# Autodesk Inventor assembly: M - Climber
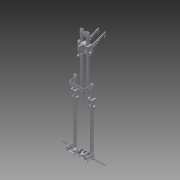
[picture p0: Inventor's stored thumbnail of the model, 180x180]
Saved by Autodesk Inventor 2013 (Build 170138000, 138)
## iProperties
Created: 2013-02-17
Part Number: M - Climber
Document SubType Name: Assembly
Designer: Moses
Mass: 5405.91 g
Surface Area: 9929.51 cm^2
Volume: 1509.49 cm^3
Density: 3.58127 g/cm^3
Author: Moses
## Documents named in this file (6)
- C:\Users\Moses\Documents\GitHub\frc2013CAD\M-Climber\M - Climber.iam
- C:\Users\Moses\Documents\GitHub\frc2013CAD\M-Climber\M - Climber Lower Rails.iam
- C:\Users\Moses\Documents\GitHub\frc2013CAD\M-Climber\M - Climber Upper Rails.iam
- C:\Users\Moses\Documents\GitHub\frc2013CAD\M-Climber\M - Carriage.iam
- C:\Users\Moses\Documents\GitHub\frc2013CAD\M-Climber\rough pulley.ipt
- C:\Users\Moses\Documents\GitHub\frc2013CAD\M-Climber\M - 18 inch shaft.ipt
## Components (8 placed, 5 different names)
1. M - Climber Lower Rails:1 [sub-assembly] — Mate:1, Flush:1, Mate:2, Tangent:1, Tangent:2, Mate:3, Tangent:3, Tangent:4, Mate:4, Mate:5, Flush:4, Mate:9
2. M - Climber Upper Rails:1 [sub-assembly] — Mate:1, Flush:1, Flush:3, Flush:6, Flush:7
3. M - Carriage:1 [sub-assembly] — Mate:2, Tangent:1, Tangent:2, Flush:2, Flush:3, Mate:9
4. M - Carriage:2 [sub-assembly] — Flush:2, Mate:3, Tangent:3, Tangent:4
5. M - 18 inch shaft:1 — Mate:4, Mate:5, Flush:4, Mate:6, Mate:7, Mate:8, Flush:5
6. rough pulley:1 — Mate:6, Flush:6
7. rough pulley:2 — Mate:7, Flush:5
8. rough pulley:3 — Mate:8, Flush:7
## Relationships (20: Mate 9, Flush 7, Tangent 4)
- Mate:1 (31.75 mm): M - Climber Lower Rails:1 ↔ M - Climber Upper Rails:1
- Flush:1 (12.7 mm): M - Climber Lower Rails:1 ↔ M - Climber Upper Rails:1
- Mate:2: M - Climber Lower Rails:1 ↔ M - Carriage:1
- Tangent:1: M - Climber Lower Rails:1 ↔ M - Carriage:1
- Tangent:2: M - Climber Lower Rails:1 ↔ M - Carriage:1
- Flush:2: M - Carriage:1 ↔ M - Carriage:2
- Mate:3: M - Climber Lower Rails:1 ↔ M - Carriage:2
- Tangent:3: M - Climber Lower Rails:1 ↔ M - Carriage:2
- Tangent:4: M - Climber Lower Rails:1 ↔ M - Carriage:2
- Flush:3: M - Climber Upper Rails:1 ↔ M - Carriage:1
- Mate:4: M - Climber Lower Rails:1 ↔ M - 18 inch shaft:1
- Mate:5: M - Climber Lower Rails:1 ↔ M - 18 inch shaft:1
- Flush:4 (-123.825 mm): M - Climber Lower Rails:1 ↔ M - 18 inch shaft:1
- Mate:6: M - 18 inch shaft:1 ↔ rough pulley:1
- Mate:7: M - 18 inch shaft:1 ↔ rough pulley:2
- Mate:8: M - 18 inch shaft:1 ↔ rough pulley:3
- Flush:5 (218.2812 mm): M - 18 inch shaft:1 ↔ rough pulley:2
- Flush:6: M - Climber Upper Rails:1 ↔ rough pulley:1
- Flush:7: M - Climber Upper Rails:1 ↔ rough pulley:3
- Mate:9 (406.4 mm): M - Climber Lower Rails:1 ↔ M - Carriage:1
